# Autodesk Inventor assembly: REAR ASSEMBLY
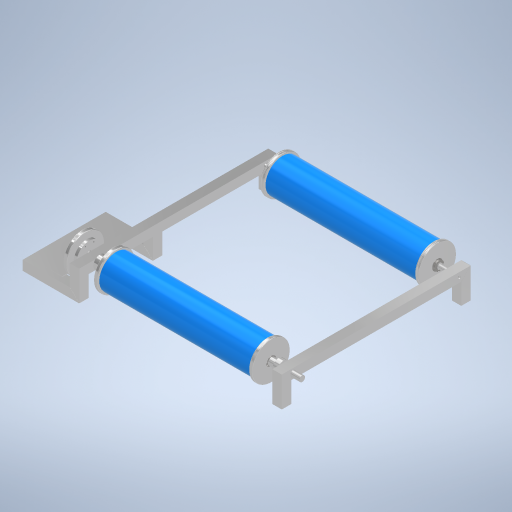
[picture p0: Inventor's stored thumbnail of the model, 512x512]
Saved by Autodesk Inventor 2023 (Build 270158000, 158)
## iProperties
Created: 2022-08-29
Part Number: REAR ASSEMBLY
Document SubType Name: Assembly
Designer: D.C. Eksteen
Author: D.C. Eksteen
## Documents named in this file (5)
- C:\Users\dylan\Desktop\Skripsie-2022\Design\CAD\REAR ASSEMBLY.iam
- C:\Users\dylan\Desktop\Skripsie-2022\Design\CAD\IDLE ROLLER.iam
- C:\Users\dylan\Desktop\Skripsie-2022\Design\CAD\POWER SHAFT ASSEMBLY.iam
- C:\Users\dylan\Desktop\Skripsie-2022\Design\CAD\LEFT FRAME.iam
- C:\Users\dylan\Desktop\Skripsie-2022\Design\CAD\RIGHT FRAME.iam
## Components (4 placed, 4 different names)
1. POWER SHAFT ASSEMBLY:1 [sub-assembly]
2. RIGHT FRAME:2 [sub-assembly]
3. LEFT FRAME:3 [sub-assembly]
4. IDLE ROLLER:1 [sub-assembly]
## Relationships (7: Mate 7)
- [Mate]: POWER SHAFT ASSEMBLY:1 ↔ RIGHT FRAME:2
- [Mate]: POWER SHAFT ASSEMBLY:1 ↔ RIGHT FRAME:2
- [Mate]: LEFT FRAME:3 ↔ IDLE ROLLER:1
- [Mate]: RIGHT FRAME:2 ↔ IDLE ROLLER:1
- [Mate]: LEFT FRAME:3 ↔ IDLE ROLLER:1
- [Mate]: RIGHT FRAME:2 ↔ IDLE ROLLER:1
- [Mate]: POWER SHAFT ASSEMBLY:1 ↔ LEFT FRAME:3
